# Autodesk Inventor assembly: Tetrix_739092
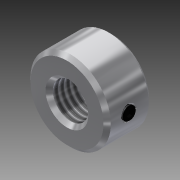
[picture p0: Inventor's stored thumbnail of the model, 180x180]
Saved by Autodesk Inventor 2015 SP1 (Build 190203100, 203)
## iProperties
Category: Collars
Company: Autodesk Inc.
Created: 2014-11-19
Part Number: Tetrix_739092
Document SubType Name: Assembly
Designer: Tetrix
Catalog Web Link: http://www.tetrixrobotics.com/TETRIX_Axle_Set_Collars
Vendor: Tetrix
Author: Autodesk Inc.
## Documents named in this file (3)
- D:\Data Folder\FTC 2015\KOP\Tetrix\Tetrix_739092.iam
- D:\Data Folder\FTC 2015\KOP\Tetrix\Tetrix_739092_Collar.ipt
- D:\Data Folder\FTC 2015\KOP\Tetrix\Tetrix_739092_Screw.ipt
## Components (2 placed, 2 different names)
1. Tetrix_739092_Collar — Mate:1
2. Tetrix_739092_Screw — Mate:1
## Relationships (1: Mate 1)
- Mate:1: Tetrix_739092_Collar ↔ Tetrix_739092_Screw
